# Autodesk Inventor assembly: full
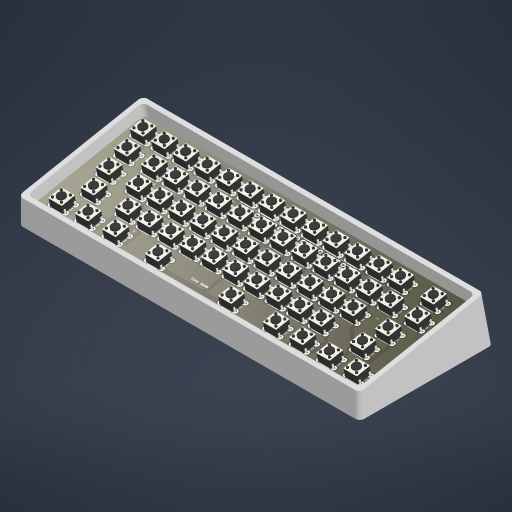
[picture p0: Inventor's stored thumbnail of the model, 512x512]
Saved by Autodesk Inventor 2024.2 (Build 282272000, 272)
## iProperties
Created: 2024-12-04
Part Number: full
Document SubType Name: Assembly
Designer: Moe
Author: Moe
## Documents named in this file (4)
- D:\Code\git\tiny-keeb\case\full.iam
- D:\Code\git\tiny-keeb\case\housing.ipt
- D:\Code\git\tiny-keeb\case\pcb fill in\pcb.ipt
- D:\Code\git\tiny-keeb\case\references\Raspberry Pi Pico-R3.ipt
## Components (3 placed, 3 different names)
1. housing:1 — Mate:1, Mate:2, Mate:3
2. pcb:1 — Mate:1, Mate:2, Mate:3
3. Raspberry Pi Pico-R3:1
## Relationships (3: Mate 3)
- Mate:1: housing:1 ↔ pcb:1
- Mate:2: housing:1 ↔ pcb:1
- Mate:3: housing:1 ↔ pcb:1
